# Autodesk Inventor assembly: KosselCNC1515_Vertex_Upper
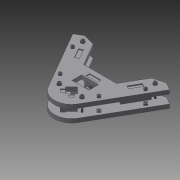
[picture p0: Inventor's stored thumbnail of the model, 180x180]
Saved by Autodesk Inventor 2014 (Build 180170000, 170)
## iProperties
Created: 2014-09-19
Part Number: KosselCNC1515_Vertex_Upper
Document SubType Name: Assembly
Designer: ThatOtherGuy
Author: ThatOtherGuy
## Documents named in this file (14)
- C:\Users\ThatOtherGuy\Documents\Inventor\KosselCNC1515\Frame\KosselCNC1515_Vertex_Upper.iam
- C:\Users\ThatOtherGuy\Documents\Inventor\KosselCNC1515\Frame\Frame_Upper_Vertical_Plate_A.ipt
- C:\Users\ThatOtherGuy\Documents\Inventor\KosselCNC1515\Frame\Frame_Upper_Vertical_Plate_B.ipt
- C:\Users\ThatOtherGuy\Documents\Inventor\KosselCNC1515\Frame\Frame_Upper_Vertical_Plate_C.ipt
- C:\Users\ThatOtherGuy\Documents\Inventor\KosselCNC1515\Frame\Frame_Upper_Plate_Pulley_A.ipt
- C:\Users\ThatOtherGuy\Documents\Inventor\KosselCNC1515\Frame\Frame_Upper_Plate_Pulley_B.ipt
- C:\Users\ThatOtherGuy\Documents\Inventor\Content Center Files\R2014\en-US\DIN 125-1  A\DIN 125 - A 3.2.ipt
- C:\Users\ThatOtherGuy\Documents\Inventor\Content Center Files\R2014\en-US\ANSI B18.3.1M(1)\ANSI B18.3.1M - M3x0.5 x 30(2).ipt
- C:\Users\ThatOtherGuy\Documents\Inventor\Content Center Files\R2014\en-US\ISO 10511\ISO 10511 - M3.ipt
- C:\Users\ThatOtherGuy\Documents\Inventor\Content Center Files\R2014\en-US\Flanged Double Shielded (Metric)\Flanged 3x10x4-2Z.ipt
- C:\Users\ThatOtherGuy\Documents\Inventor\KosselCNC1515\Frame\Frame_Upper_Plate_Bottom.ipt
- C:\Users\ThatOtherGuy\Documents\Inventor\Content Center Files\R2014\en-US\ANSI B18.3.1M(1)\ANSI B18.3.1M - M3x0.5 x 10(2).ipt
- C:\Users\ThatOtherGuy\Documents\Inventor\Content Center Files\R2014\en-US\ANSI B18.3.1M(1)\ANSI B18.3.1M - M3x0.5 x 35(2).ipt
- C:\Users\ThatOtherGuy\Documents\Inventor\Content Center Files\R2014\en-US\DIN 562\DIN 562 - M3 x 5.5.ipt
## Components (61 placed, 14 different names)
1. Frame_Upper_Plate_Bottom:1 — Mate:1, Mate:2, Mate:3, Mate:4, Mate:5, Mate:6, Mate:7, Mate:8, Mate:9, Mate:10, Mate:11, Mate:12, Mate:16, Mate:17, Mate:18, Mate:20, Insert:16, Insert:17, Insert:18, Insert:19, Insert:24, Insert:25, Insert:26, Insert:27, Insert:39, Insert:40, Insert:41, Insert:42
2. Frame_Upper_Plate_Bottom:2 — Mate:13, Mate:14, Mate:15, Insert:12, Insert:13, Insert:14, Insert:15, Insert:20, Insert:21, Insert:22, Insert:23, Mate:36, Insert:31, Insert:36, Insert:37, Insert:38
3. Frame_Upper_Vertical_Plate_A:1 — Mate:1, Mate:2, Mate:3, Insert:48, Insert:49
4. Frame_Upper_Vertical_Plate_B:1 — Mate:4, Mate:5, Mate:6, Insert:47, Insert:50
5. Frame_Upper_Vertical_Plate_C:1 — Mate:7, Mate:8, Mate:9, Mate:14
6. Frame_Lower_Vertical_Plate_C:2 — Mate:10, Mate:11, Mate:12, Mate:13, Mate:15
7. Frame_Upper_Plate_Pulley_A:1 — Mate:16, Mate:17, Mate:18, Mate:19, Flush:1, Insert:1, Insert:2, Mate:21
8. Frame_Upper_Plate_Pulley_B:1 — Mate:19, Flush:1, Mate:20
9. DIN 125-1 A A 3.2:1 — Insert:1, Mate:22
10. DIN 125-1 A A 3.2:2 — Insert:2, Insert:3
11. DIN 125-1 A A 3.2:3 — Insert:3, Insert:4
12. DIN 125-1 A A 3.2:4 — Insert:4, Insert:5
13. DIN 125-1 A A 3.2:5 — Insert:5, Insert:6
14. DIN 125-1 A A 3.2:6 — Insert:6, Insert:7
15. DIN 125-1 A A 3.2:7 — Insert:7, Insert:8
16. DIN 125-1 A A 3.2:8 — Insert:8, Insert:9
17. Broached Socket Head Cap Screw - Metric M3x0.5 x 30:1 — Mate:21, Mate:22, Mate:28, Mate:32, Mate:34
18. DIN 125-1 A A 3.2:9 — Insert:9, Insert:10
19. DIN 125-1 A A 3.2:10 — Insert:10, Insert:11
20. DIN 125-1 A A 3.2:11 — Insert:11, Mate:33
21. DIN 125-1 A A 3.2:12 — Mate:29
22. DIN EN ISO 10511 M3:1 — Mate:28, Mate:29
23. Flanged Double Shielded (Metric) 3-10-4:1 — Mate:30, Mate:31, Mate:32, Mate:33
24. Flanged Double Shielded (Metric) 3-10-4:2 — Mate:30, Mate:31, Mate:35
25. DIN EN ISO 10511 M3:2 — Mate:34, Mate:35
26. DIN 125-1 A A 3.2:13 — Insert:12, Mate:37
27. DIN 125-1 A A 3.2:14 — Insert:13, Insert:28
28. DIN 125-1 A A 3.2:15 — Insert:14, Insert:30
29. DIN 125-1 A A 3.2:16 — Insert:15, Insert:29
30. DIN 125-1 A A 3.2:17 — Insert:16, Insert:45
31. DIN 125-1 A A 3.2:18 — Insert:17, Insert:46
32. DIN 125-1 A A 3.2:19 — Insert:18, Insert:43
33. DIN 125-1 A A 3.2:20 — Insert:19, Insert:44
34. Broached Socket Head Cap Screw - Metric M3x0.5 x 10:1 — Insert:20
35. Broached Socket Head Cap Screw - Metric M3x0.5 x 10:2 — Insert:21
36. Broached Socket Head Cap Screw - Metric M3x0.5 x 10:3 — Insert:22
37. Broached Socket Head Cap Screw - Metric M3x0.5 x 10:4 — Insert:23
38. Broached Socket Head Cap Screw - Metric M3x0.5 x 10:5 — Insert:24
39. Broached Socket Head Cap Screw - Metric M3x0.5 x 10:6 — Insert:25
40. Broached Socket Head Cap Screw - Metric M3x0.5 x 10:7 — Insert:26
41. Broached Socket Head Cap Screw - Metric M3x0.5 x 10:8 — Insert:27
42. Broached Socket Head Cap Screw - Metric M3x0.5 x 35:1 — Mate:36, Mate:37
43. Broached Socket Head Cap Screw - Metric M3x0.5 x 35:2 — Insert:28
44. Broached Socket Head Cap Screw - Metric M3x0.5 x 35:3 — Insert:29
45. Broached Socket Head Cap Screw - Metric M3x0.5 x 35:4 — Insert:30
46. DIN 562 M3:1 — Insert:31
47. DIN 562 M3:6 — Insert:36
48. DIN 562 M3:7 — Insert:37
49. DIN 562 M3:8 — Insert:38
50. DIN 562 M3:9 — Insert:39
51. DIN 562 M3:10 — Insert:40
52. DIN 562 M3:11 — Insert:41
53. DIN 562 M3:12 — Insert:42
54. DIN EN ISO 10511 M3:3 — Insert:43
55. DIN EN ISO 10511 M3:4 — Insert:44
56. DIN EN ISO 10511 M3:5 — Insert:45
57. DIN EN ISO 10511 M3:6 — Insert:46
58. Broached Socket Head Cap Screw - Metric M3x0.5 x 10:9 — Insert:47
59. Broached Socket Head Cap Screw - Metric M3x0.5 x 10:10 — Insert:48
60. DIN 562 M3:13 — Insert:49
61. DIN 562 M3:14 — Insert:50
## Relationships (79: Insert 46, Mate 32, Flush 1)
- Mate:1: Frame_Upper_Plate_Bottom:1 ↔ Frame_Upper_Vertical_Plate_A:1
- Mate:2: Frame_Upper_Plate_Bottom:1 ↔ Frame_Upper_Vertical_Plate_A:1
- Mate:3: Frame_Upper_Plate_Bottom:1 ↔ Frame_Upper_Vertical_Plate_A:1
- Mate:4: Frame_Upper_Plate_Bottom:1 ↔ Frame_Upper_Vertical_Plate_B:1
- Mate:5: Frame_Upper_Plate_Bottom:1 ↔ Frame_Upper_Vertical_Plate_B:1
- Mate:6: Frame_Upper_Plate_Bottom:1 ↔ Frame_Upper_Vertical_Plate_B:1
- Mate:7: Frame_Upper_Plate_Bottom:1 ↔ Frame_Upper_Vertical_Plate_C:1
- Mate:8: Frame_Upper_Plate_Bottom:1 ↔ Frame_Upper_Vertical_Plate_C:1
- Mate:9: Frame_Upper_Plate_Bottom:1 ↔ Frame_Upper_Vertical_Plate_C:1
- Mate:10: Frame_Upper_Plate_Bottom:1 ↔ Frame_Lower_Vertical_Plate_C:2
- Mate:11: Frame_Upper_Plate_Bottom:1 ↔ Frame_Lower_Vertical_Plate_C:2
- Mate:12: Frame_Upper_Plate_Bottom:1 ↔ Frame_Lower_Vertical_Plate_C:2
- Mate:13: Frame_Upper_Plate_Bottom:2 ↔ Frame_Lower_Vertical_Plate_C:2
- Mate:14: Frame_Upper_Plate_Bottom:2 ↔ Frame_Upper_Vertical_Plate_C:1
- Mate:15: Frame_Upper_Plate_Bottom:2 ↔ Frame_Lower_Vertical_Plate_C:2
- Mate:16: Frame_Upper_Plate_Bottom:1 ↔ Frame_Upper_Plate_Pulley_A:1
- Mate:17: Frame_Upper_Plate_Bottom:1 ↔ Frame_Upper_Plate_Pulley_A:1
- Mate:18: Frame_Upper_Plate_Bottom:1 ↔ Frame_Upper_Plate_Pulley_A:1
- Mate:19: Frame_Upper_Plate_Pulley_A:1 ↔ Frame_Upper_Plate_Pulley_B:1
- Flush:1: Frame_Upper_Plate_Pulley_A:1 ↔ Frame_Upper_Plate_Pulley_B:1
- Mate:20: Frame_Upper_Plate_Bottom:1 ↔ Frame_Upper_Plate_Pulley_B:1
- Insert:1: Frame_Upper_Plate_Pulley_A:1 ↔ DIN 125-1 A A 3.2:1
- Insert:2: Frame_Upper_Plate_Pulley_A:1 ↔ DIN 125-1 A A 3.2:2
- Insert:3: DIN 125-1 A A 3.2:2 ↔ DIN 125-1 A A 3.2:3
- Insert:4: DIN 125-1 A A 3.2:3 ↔ DIN 125-1 A A 3.2:4
- Insert:5: DIN 125-1 A A 3.2:4 ↔ DIN 125-1 A A 3.2:5
- Insert:6: DIN 125-1 A A 3.2:5 ↔ DIN 125-1 A A 3.2:6
- Insert:7: DIN 125-1 A A 3.2:6 ↔ DIN 125-1 A A 3.2:7
- Insert:8: DIN 125-1 A A 3.2:7 ↔ DIN 125-1 A A 3.2:8
- Mate:21: Frame_Upper_Plate_Pulley_A:1 ↔ Broached Socket Head Cap Screw - Metric M3x0.5 x 30:1
- Mate:22: DIN 125-1 A A 3.2:1 ↔ Broached Socket Head Cap Screw - Metric M3x0.5 x 30:1
- Insert:9: DIN 125-1 A A 3.2:8 ↔ DIN 125-1 A A 3.2:9
- Insert:10: DIN 125-1 A A 3.2:9 ↔ DIN 125-1 A A 3.2:10
- Insert:11: DIN 125-1 A A 3.2:10 ↔ DIN 125-1 A A 3.2:11
- Mate:28: Broached Socket Head Cap Screw - Metric M3x0.5 x 30:1 ↔ DIN EN ISO 10511 M3:1
- Mate:29: DIN 125-1 A A 3.2:12 ↔ DIN EN ISO 10511 M3:1
- Mate:30: Flanged Double Shielded (Metric) 3-10-4:1 ↔ Flanged Double Shielded (Metric) 3-10-4:2
- Mate:31: Flanged Double Shielded (Metric) 3-10-4:1 ↔ Flanged Double Shielded (Metric) 3-10-4:2
- Mate:32: Broached Socket Head Cap Screw - Metric M3x0.5 x 30:1 ↔ Flanged Double Shielded (Metric) 3-10-4:1
- Mate:33: DIN 125-1 A A 3.2:11 ↔ Flanged Double Shielded (Metric) 3-10-4:1
- Mate:34: Broached Socket Head Cap Screw - Metric M3x0.5 x 30:1 ↔ DIN EN ISO 10511 M3:2
- Mate:35: Flanged Double Shielded (Metric) 3-10-4:2 ↔ DIN EN ISO 10511 M3:2
- Insert:12: Frame_Upper_Plate_Bottom:2 ↔ DIN 125-1 A A 3.2:13
- Insert:13: Frame_Upper_Plate_Bottom:2 ↔ DIN 125-1 A A 3.2:14
- Insert:14: Frame_Upper_Plate_Bottom:2 ↔ DIN 125-1 A A 3.2:15
- Insert:15: Frame_Upper_Plate_Bottom:2 ↔ DIN 125-1 A A 3.2:16
- Insert:16: Frame_Upper_Plate_Bottom:1 ↔ DIN 125-1 A A 3.2:17
- Insert:17: Frame_Upper_Plate_Bottom:1 ↔ DIN 125-1 A A 3.2:18
- Insert:18: Frame_Upper_Plate_Bottom:1 ↔ DIN 125-1 A A 3.2:19
- Insert:19: Frame_Upper_Plate_Bottom:1 ↔ DIN 125-1 A A 3.2:20
- Insert:20: Frame_Upper_Plate_Bottom:2 ↔ Broached Socket Head Cap Screw - Metric M3x0.5 x 10:1
- Insert:21: Frame_Upper_Plate_Bottom:2 ↔ Broached Socket Head Cap Screw - Metric M3x0.5 x 10:2
- Insert:22: Frame_Upper_Plate_Bottom:2 ↔ Broached Socket Head Cap Screw - Metric M3x0.5 x 10:3
- Insert:23: Frame_Upper_Plate_Bottom:2 ↔ Broached Socket Head Cap Screw - Metric M3x0.5 x 10:4
- Insert:24: Frame_Upper_Plate_Bottom:1 ↔ Broached Socket Head Cap Screw - Metric M3x0.5 x 10:5
- Insert:25: Frame_Upper_Plate_Bottom:1 ↔ Broached Socket Head Cap Screw - Metric M3x0.5 x 10:6
- Insert:26: Frame_Upper_Plate_Bottom:1 ↔ Broached Socket Head Cap Screw - Metric M3x0.5 x 10:7
- Insert:27: Frame_Upper_Plate_Bottom:1 ↔ Broached Socket Head Cap Screw - Metric M3x0.5 x 10:8
- Mate:36: Frame_Upper_Plate_Bottom:2 ↔ Broached Socket Head Cap Screw - Metric M3x0.5 x 35:1
- Mate:37: DIN 125-1 A A 3.2:13 ↔ Broached Socket Head Cap Screw - Metric M3x0.5 x 35:1
- Insert:28: DIN 125-1 A A 3.2:14 ↔ Broached Socket Head Cap Screw - Metric M3x0.5 x 35:2
- Insert:29: DIN 125-1 A A 3.2:16 ↔ Broached Socket Head Cap Screw - Metric M3x0.5 x 35:3
- Insert:30: DIN 125-1 A A 3.2:15 ↔ Broached Socket Head Cap Screw - Metric M3x0.5 x 35:4
- Insert:31: Frame_Upper_Plate_Bottom:2 ↔ DIN 562 M3:1
- Insert:36: Frame_Upper_Plate_Bottom:2 ↔ DIN 562 M3:6
- Insert:37: Frame_Upper_Plate_Bottom:2 ↔ DIN 562 M3:7
- Insert:38: Frame_Upper_Plate_Bottom:2 ↔ DIN 562 M3:8
- Insert:39: Frame_Upper_Plate_Bottom:1 ↔ DIN 562 M3:9
- Insert:40: Frame_Upper_Plate_Bottom:1 ↔ DIN 562 M3:10
- Insert:41: Frame_Upper_Plate_Bottom:1 ↔ DIN 562 M3:11
- Insert:42: Frame_Upper_Plate_Bottom:1 ↔ DIN 562 M3:12
- Insert:43: DIN 125-1 A A 3.2:19 ↔ DIN EN ISO 10511 M3:3
- Insert:44: DIN 125-1 A A 3.2:20 ↔ DIN EN ISO 10511 M3:4
- Insert:45: DIN 125-1 A A 3.2:17 ↔ DIN EN ISO 10511 M3:5
- Insert:46: DIN 125-1 A A 3.2:18 ↔ DIN EN ISO 10511 M3:6
- Insert:47: Frame_Upper_Vertical_Plate_B:1 ↔ Broached Socket Head Cap Screw - Metric M3x0.5 x 10:9
- Insert:48: Frame_Upper_Vertical_Plate_A:1 ↔ Broached Socket Head Cap Screw - Metric M3x0.5 x 10:10
- Insert:49: Frame_Upper_Vertical_Plate_A:1 ↔ DIN 562 M3:13
- Insert:50: Frame_Upper_Vertical_Plate_B:1 ↔ DIN 562 M3:14
